# Autodesk Inventor assembly: Assembly1
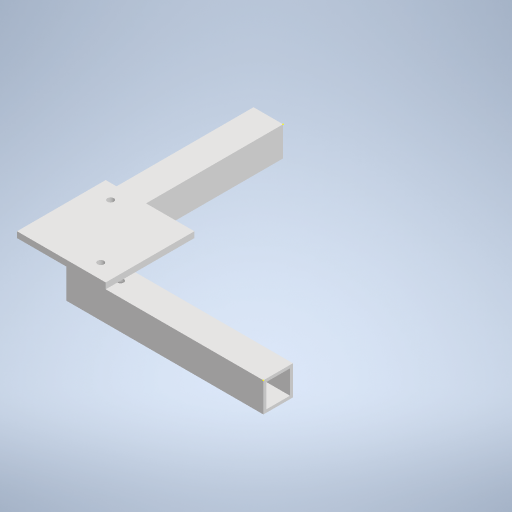
[picture p0: Inventor's stored thumbnail of the model, 512x512]
Saved by Autodesk Inventor 2023 (Build 270158000, 158)
## iProperties
Created: 2022-04-25
Part Number: Assembly1
Document SubType Name: Assembly
Designer: yuta
Author: yuta
## Documents named in this file (3)
- C:\Users\yuta\Documents\NHK\Assembly1.iam
- C:\Users\yuta\Documents\NHK\Part1.ipt
- C:\Users\yuta\Documents\NHK\Part2.ipt
## Components (3 placed, 2 different names)
1. Part1:1 — メイト:1, メイト:2
2. Part1:2 — メイト:3, メイト:4
3. Part2:1 — メイト:1, メイト:2, メイト:3, メイト:4
## Relationships (4: Mate 4)
- メイト:1 [Mate]: Part1:1 ↔ Part2:1
- メイト:2 [Mate]: Part1:1 ↔ Part2:1
- メイト:3 [Mate]: Part1:2 ↔ Part2:1
- メイト:4 [Mate]: Part1:2 ↔ Part2:1
